# Autodesk Inventor assembly: Gyro Assmebly
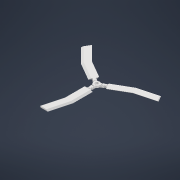
[picture p0: Inventor's stored thumbnail of the model, 180x180]
Saved by Autodesk Inventor 2022 (Build 260153000, 153)
## iProperties
Created: 2021-12-15
Part Number: Gyro Assmebly
Document SubType Name: Assembly
Designer: Wilson
Author: Wilson
## Documents named in this file (3)
- C:\Users\Wilson\OneDrive\Documents\Projekts\Rocketery\Rocketery\Rocket Designs\Gyro Assmebly.iam
- C:\Users\Wilson\OneDrive\Documents\Projekts\Rocketery\CAD Files v1\Rocoverey System Gyro\Aerospace\Gyrocopter Base.ipt
- C:\Users\Wilson\OneDrive\Documents\Projekts\Rocketery\CAD Files v1\Rocoverey System Gyro\Aerospace\Gyrocopter Blade.ipt
## Components (4 placed, 2 different names)
1. Gyrocopter Base:1 — Mate:1, Mate:2, Mate:3, Mate:4, Mate:5, Mate:6
2. Gyrocopter Blade:1 — Mate:1, Mate:2, Angle:1, Angle:3
3. Gyrocopter Blade:2 — Mate:3, Mate:5, Angle:1, Angle:2
4. Gyrocopter Blade:3 — Mate:4, Mate:6, Angle:2, Angle:3
## Relationships (9: Mate 6, Angle 3)
- Mate:1: Gyrocopter Base:1 ↔ Gyrocopter Blade:1
- Mate:2: Gyrocopter Base:1 ↔ Gyrocopter Blade:1
- Mate:3: Gyrocopter Base:1 ↔ Gyrocopter Blade:2
- Mate:4: Gyrocopter Base:1 ↔ Gyrocopter Blade:3
- Mate:5: Gyrocopter Base:1 ↔ Gyrocopter Blade:2
- Mate:6: Gyrocopter Base:1 ↔ Gyrocopter Blade:3
- Angle:1 (0 deg): Gyrocopter Blade:1 ↔ Gyrocopter Blade:2
- Angle:2 (0 deg): Gyrocopter Blade:2 ↔ Gyrocopter Blade:3
- Angle:3 (0 deg): Gyrocopter Blade:1 ↔ Gyrocopter Blade:3
